# Autodesk Inventor assembly: Stepper-D15-S18_asm
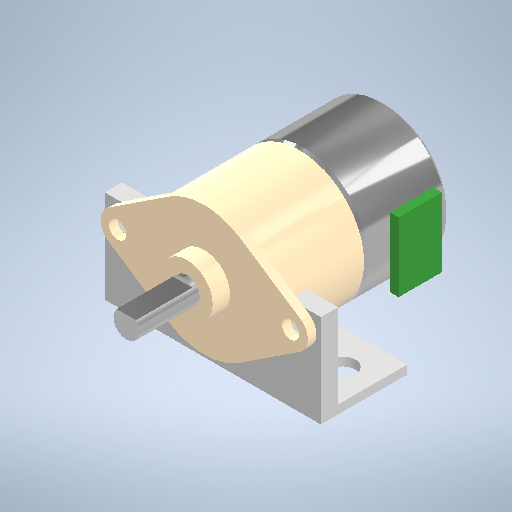
[picture p0: Inventor's stored thumbnail of the model, 512x512]
Saved by Autodesk Inventor 2025.3 (Build 293356000, 356)
## iProperties
Created: 2025-06-27
Part Number: Stepper-D15-S18_asm
Document SubType Name: Assembly
Designer: yamashita1
Author: yamashita1
## Documents named in this file (3)
- G:\マイドライブ\project\micro-mouse\3D-Model\Stepper-D15-S18_asm.iam
- G:\マイドライブ\project\micro-mouse\3D-Model\Stepper-D15-S18_Braket.ipt
- G:\マイドライブ\project\micro-mouse\3D-Model\Stepper-D15-S18.ipt
## Components (2 placed, 2 different names)
1. Stepper-D15-S18_Braket:1 — メイト:2, メイト:3, メイト:4
2. Stepper-D15-S18:1 — メイト:2, メイト:3, メイト:4
## Relationships (3: Mate 3)
- メイト:2 [Mate]: Stepper-D15-S18_Braket:1 ↔ Stepper-D15-S18:1
- メイト:3 [Mate]: Stepper-D15-S18_Braket:1 ↔ Stepper-D15-S18:1
- メイト:4 [Mate]: Stepper-D15-S18_Braket:1 ↔ Stepper-D15-S18:1
